# Autodesk Inventor assembly: current_sensor
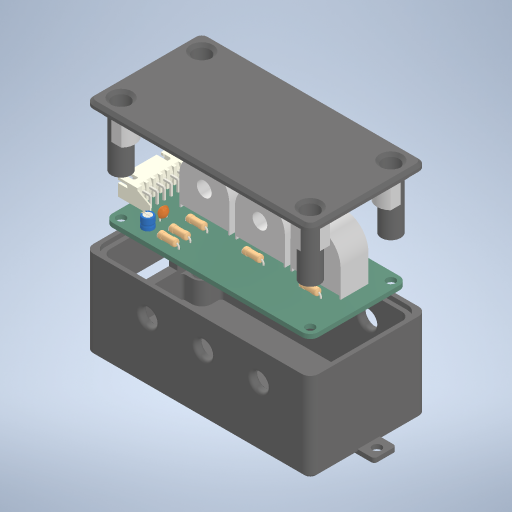
[picture p0: Inventor's stored thumbnail of the model, 512x512]
Saved by Autodesk Inventor 2023 (Build 270158000, 158)
## iProperties
Created: 2023-10-27
Part Number: current_sensor
Document SubType Name: Assembly
Designer: mark
Author: mark
## Documents named in this file (4)
- D:\Egyetem\BME MSc\Diplomamunka\opendaq\cad\current sensor\current_sensor.iam
- D:\Egyetem\BME MSc\Diplomamunka\opendaq\cad\current sensor\current_sensor_base.ipt
- D:\Egyetem\BME MSc\Diplomamunka\opendaq\pcb\zmct_3phase\zmct_3phase\zmct_3phase.iam
- D:\Egyetem\BME MSc\Diplomamunka\opendaq\cad\current sensor\current_sensor_cover.ipt
## Components (3 placed, 3 different names)
1. current_sensor_base:1 — Mate:1, Mate:2, Mate:6, Mate:7, Mate:8, Mate:9
2. zmct_3phase:1 [sub-assembly] — Mate:1, Mate:2, Mate:9
3. current_sensor_cover:1 — Mate:6, Mate:7, Mate:8
## Relationships (6: Mate 6)
- Mate:1: current_sensor_base:1 ↔ zmct_3phase:1
- Mate:2: current_sensor_base:1 ↔ zmct_3phase:1
- Mate:6 (45 mm): current_sensor_base:1 ↔ current_sensor_cover:1
- Mate:7: current_sensor_base:1 ↔ current_sensor_cover:1
- Mate:8: current_sensor_base:1 ↔ current_sensor_cover:1
- Mate:9 (30 mm): current_sensor_base:1 ↔ zmct_3phase:1
